# Autodesk Inventor assembly: Assembly8
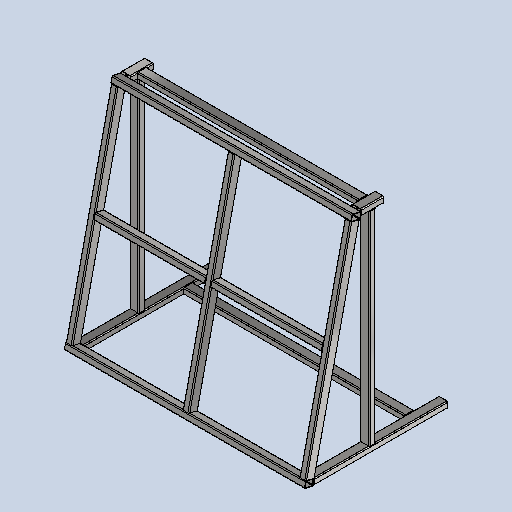
[picture p0: Inventor's stored thumbnail of the model, 512x512]
Saved by Autodesk Inventor 2025 (Build 290162010, 162A)
## iProperties
Created: 2024-09-20
Part Number: Assembly8
Document SubType Name: Assembly
Designer: admin
Author: admin
## Documents named in this file (5)
- C:\Users\admin\YandexDisk-badmisterfox\домашниий пк\Inventor\BSH_Beshkino_bio_tank\Assembly8.iam
- C:\Users\admin\YandexDisk-badmisterfox\домашниий пк\Inventor\BSH_Beshkino_bio_tank\Тумба 3.iam
- C:\Users\admin\YandexDisk-badmisterfox\домашниий пк\Inventor\BSH_Beshkino_bio_tank\Нога тумба 3.1.iam
- C:\Users\admin\YandexDisk-badmisterfox\домашниий пк\Inventor\BSH_Beshkino_bio_tank\Нога тумба 3.2.iam
- C:\Users\admin\YandexDisk-badmisterfox\домашниий пк\Inventor\BSH_Beshkino_bio_tank\ISO 4019 - 60x40x3 - 1286,407.ipt
## Components (5 placed, 4 different names)
1. Тумба 3:1 [sub-assembly]
2. Нога тумба 3.1:1 [sub-assembly]
3. Нога тумба 3.2:1 [sub-assembly]
4. ISO 4019 - 60x40x3 - 1286,407:1
5. ISO 4019 - 60x40x3 - 1286,407:2
## Relationships (13: Flush 7, Mate 6)
- [Mate]: Нога тумба 3.2:1 ↔ ISO 4019 - 60x40x3 - 1286,407:1
- [Flush]: Нога тумба 3.2:1 ↔ ISO 4019 - 60x40x3 - 1286,407:1
- [Flush] (50 mm): Нога тумба 3.2:1 ↔ ISO 4019 - 60x40x3 - 1286,407:1
- [Mate]: Нога тумба 3.2:1 ↔ ISO 4019 - 60x40x3 - 1286,407:2
- [Flush]: Нога тумба 3.2:1 ↔ ISO 4019 - 60x40x3 - 1286,407:2
- [Flush] (50 mm): Нога тумба 3.2:1 ↔ ISO 4019 - 60x40x3 - 1286,407:2
- [Mate] (1270 mm): Нога тумба 3.1:1 ↔ Нога тумба 3.2:1
- [Flush]: Нога тумба 3.1:1 ↔ Нога тумба 3.2:1
- [Flush] (-400 mm): Нога тумба 3.1:1 ↔ Нога тумба 3.2:1
- [Flush]: Тумба 3:1 ↔ Нога тумба 3.1:1
- [Mate] (-10 mm): Тумба 3:1 ↔ Нога тумба 3.1:1
- [Mate] (5 mm): Тумба 3:1 ↔ Нога тумба 3.2:1
- [Mate]: Тумба 3:1 ↔ Нога тумба 3.2:1
